# Autodesk Inventor assembly: Aspa
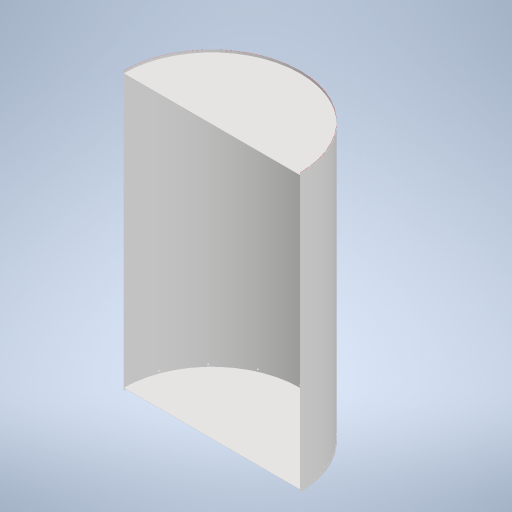
[picture p0: Inventor's stored thumbnail of the model, 512x512]
Saved by Autodesk Inventor 2024 (Build 280153000, 153)
## iProperties
Created: 2024-04-25
Part Number: Aspa
Document SubType Name: Assembly
Designer: alexa
Author: alexa
## Documents named in this file (3)
- C:\Users\alexa\OneDrive\Escritorio\Energia Eolica\Aspa.iam
- C:\Users\alexa\OneDrive\Escritorio\Energia Eolica\Aspa2.ipt
- C:\Users\alexa\OneDrive\Escritorio\Energia Eolica\Aspa1.ipt
## Components (3 placed, 2 different names)
1. Aspa2:1 — Mate:2, Mate:3
2. Aspa1:1 — Mate:1, Mate:2, Mate:3, Mate:4, Mate:5
3. Aspa2:2 — Mate:4, Mate:5
## Relationships (5: Mate 5)
- Mate:1: Aspa1:1
- Mate:2: Aspa2:1 ↔ Aspa1:1
- Mate:3: Aspa2:1 ↔ Aspa1:1
- Mate:4: Aspa1:1 ↔ Aspa2:2
- Mate:5: Aspa1:1 ↔ Aspa2:2
